# Autodesk Inventor assembly: Assembly1
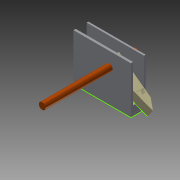
[picture p0: Inventor's stored thumbnail of the model, 180x180]
Saved by Autodesk Inventor 2015 (Build 190159000, 159)
## iProperties
Created: 2015-01-12
Part Number: Assembly1
Document SubType Name: Weldment
Designer: whitaus15
Weld Material: Welded Aluminum-6061
Author: whitaus15
## Documents named in this file (4)
- \\lhssvr02\Homedirs\Robotics Club\CAD Model 2015\Game Components\The Tote Collector-Arms\Imported Components\Assembly1.iam
- \\lhssvr02\Homedirs\Robotics Club\CAD Model 2015\Game Components\The Tote Collector-Arms\Imported Components\hook diagram.ipt
- \\lhssvr02\Homedirs\Robotics Club\CAD Model 2015\Game Components\The Tote Collector-Arms\Imported Components\hook.ipt
- \\lhssvr02\Homedirs\Robotics Club\CAD Model 2015\Game Components\The Tote Collector-Arms\Imported Components\screw.ipt
## Components (3 placed, 3 different names)
1. hook diagram:1 — Mate:1, Mate:2
2. hook:1 — Mate:1, Mate:3
3. screw:3 — Mate:2, Mate:3
## Relationships (3: Mate 3)
- Mate:1: hook diagram:1 ↔ hook:1
- Mate:2: hook diagram:1 ↔ screw:3
- Mate:3: hook:1 ↔ screw:3
